# Autodesk Inventor assembly: inside_motor_c_channel
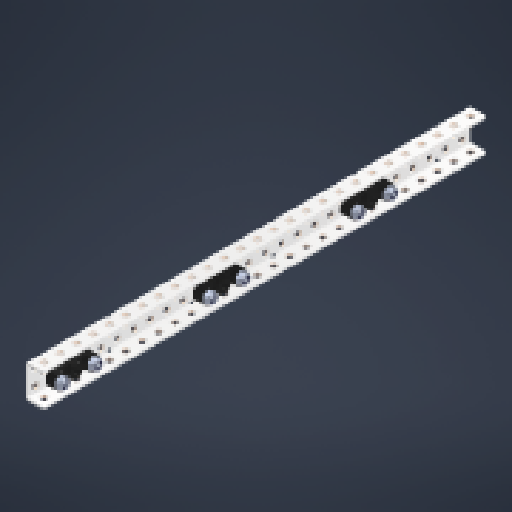
[picture p0: Inventor's stored thumbnail of the model, 512x512]
Saved by Autodesk Inventor 2023 (Build 270158000, 158)
## iProperties
Created: 2023-08-05
Part Number: inside_motor_c_channel
Document SubType Name: Assembly
Designer: srbel
Author: srbel
## Documents named in this file (6)
- C:\CAD\OverUnderCAD\Drive\inside_motor_c_channel.iam
- C:\CAD\OverUnderCAD\VEX-CAD-Inventor-1.4.0\Structure\C Channel\Aluminum 1x2x1\inside_motor_c_channel.ipt
- C:\CAD\OverUnderCAD\VEX-CAD-Inventor-1.4.0\Motion\Shaft LS\inside_motor_c_channel.ipt
- C:\CAD\OverUnderCAD\VEX-CAD-Inventor-1.4.0\Structure\Hardware\Screw Steel - Star\SScrew Star Threaded .500.ipt
- C:\CAD\OverUnderCAD\VEX-CAD-Inventor-1.4.0\Structure\Hardware\Screw Steel - Star.ipt
- C:\CAD\OverUnderCAD\VEX-CAD-Inventor-1.4.0\Structure\Hardware\inside_motor_c_channel.ipt
## Components (16 placed, 2 different names)
1. inside_motor_c_channel:1 — Insert:2, Insert:1, Insert:6, Insert:5, Insert:22, Insert:21, Insert:23, Insert:24, Insert:27, Insert:28, Insert:31, Insert:32
2. inside_motor_c_channel:2 — Insert:2, Insert:1, Insert:41, Insert:42
3. inside_motor_c_channel:4 — Insert:6, Insert:5, Insert:37, Insert:38
4. inside_motor_c_channel:6 — Insert:22, Insert:21, Insert:33, Insert:34
5. SScrew Star Threaded .500:1 — Insert:23
6. SScrew Star Threaded .500:2 — Insert:24
7. SScrew Star Threaded .500:5 — Insert:27
8. SScrew Star Threaded .500:6 — Insert:28
9. SScrew Star Threaded .500:9 — Insert:31
10. SScrew Star Threaded .500:10 — Insert:32
11. inside_motor_c_channel:7 — Insert:33
12. inside_motor_c_channel:8 — Insert:34
13. inside_motor_c_channel:11 — Insert:37
14. inside_motor_c_channel:12 — Insert:38
15. inside_motor_c_channel:15 — Insert:41
16. inside_motor_c_channel:16 — Insert:42
## Relationships (18: Insert 18)
- Insert:2: inside_motor_c_channel:1 ↔ inside_motor_c_channel:2
- Insert:1: inside_motor_c_channel:1 ↔ inside_motor_c_channel:2
- Insert:6: inside_motor_c_channel:1 ↔ inside_motor_c_channel:4
- Insert:5: inside_motor_c_channel:1 ↔ inside_motor_c_channel:4
- Insert:22: inside_motor_c_channel:1 ↔ inside_motor_c_channel:6
- Insert:21: inside_motor_c_channel:1 ↔ inside_motor_c_channel:6
- Insert:23: inside_motor_c_channel:1 ↔ SScrew Star Threaded .500:1
- Insert:24: inside_motor_c_channel:1 ↔ SScrew Star Threaded .500:2
- Insert:27: inside_motor_c_channel:1 ↔ SScrew Star Threaded .500:5
- Insert:28: inside_motor_c_channel:1 ↔ SScrew Star Threaded .500:6
- Insert:31: inside_motor_c_channel:1 ↔ SScrew Star Threaded .500:9
- Insert:32: inside_motor_c_channel:1 ↔ SScrew Star Threaded .500:10
- Insert:33: inside_motor_c_channel:6 ↔ inside_motor_c_channel:7
- Insert:34: inside_motor_c_channel:6 ↔ inside_motor_c_channel:8
- Insert:37: inside_motor_c_channel:4 ↔ inside_motor_c_channel:11
- Insert:38: inside_motor_c_channel:4 ↔ inside_motor_c_channel:12
- Insert:41: inside_motor_c_channel:2 ↔ inside_motor_c_channel:15
- Insert:42: inside_motor_c_channel:2 ↔ inside_motor_c_channel:16
